# Autodesk Inventor assembly: 560H_plus_Blumotion NL=270 mm Chipboard screws 661.1450.HG 6,3x14,5 L Top row R Top row LD drillings both
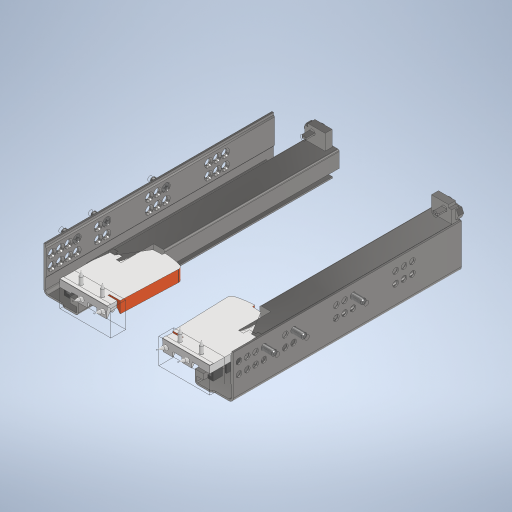
[picture p0: Inventor's stored thumbnail of the model, 512x512]
Saved by Autodesk Inventor 2024 (Build 280153000, 153)
## iProperties
Created: 2019-09-10
Part Number: 560H_plus_Blumotion NL=270 mm Chipboard screws 661.1450.HG 6,3x14,5 L Top row R Top row LD drillings both
Document SubType Name: Assembly
Designer: RokasM
Author: RokasM
## Documents named in this file (457)
- C:\W4INV 2024 Design\LIBRARY\Sliders\Blum TANDEM PLUS BLUMOTION 560 H\560H_iassembly_v2_LD.iam
- C:\W4INV 2024 Design\LIBRARY\Sliders\Blum TANDEM PLUS BLUMOTION 560 H\Blum_TANDEM_PLUS_BLUMOTION_560H.IPT
- C:\W4INV 2024 Design\LIBRARY\Sliders\Blum TANDEM PLUS BLUMOTION 560 H\Locking device.ipt
- C:\W4INV 2024 Design\LIBRARY\Sliders\Blum TANDEM PLUS BLUMOTION 560 H\Locking_device\Locking device L.ipt
- C:\W4INV 2024 Design\LIBRARY\Sliders\Blum TANDEM PLUS BLUMOTION 560 H\Locking_device\Locking device R.ipt
- C:\W4INV 2024 Design\LIBRARY\Sliders\Blum TANDEM PLUS BLUMOTION 560 H\560H\560H2700B Chipboard screws top_row L.ipt
- C:\W4INV 2024 Design\LIBRARY\Sliders\Blum TANDEM PLUS BLUMOTION 560 H\560H\560H2700B Chipboard screws top_row R.ipt
- C:\W4INV 2020 Design\LIBRARY\Rollers\Blum TANDEM PLUS BLUMOTION 560 H\Locking device.ipt
- 560H_plus_Blumotion NL=250 mm Chipboard screws 4x15 L Bottom row R Bottom row LD drillings B.iam
- 560H_plus_Blumotion NL=250 mm Chipboard screws 4x15 L Bottom row R Bottom row LD drillings both.iam
- 560H_plus_Blumotion NL=250 mm Chipboard screws 4x15 L Bottom row R Bottom row LD drillings F.iam
- 560H_plus_Blumotion NL=250 mm Chipboard screws 4x15 L Bottom row R Bottom row LD drillings none.iam
- 560H_plus_Blumotion NL=250 mm Chipboard screws 4x15 L Bottom row R Top row LD drillings B.iam
- 560H_plus_Blumotion NL=250 mm Chipboard screws 4x15 L Bottom row R Top row LD drillings both.iam
- 560H_plus_Blumotion NL=250 mm Chipboard screws 4x15 L Bottom row R Top row LD drillings F.iam
- 560H_plus_Blumotion NL=250 mm Chipboard screws 4x15 L Bottom row R Top row LD drillings none.iam
- 560H_plus_Blumotion NL=250 mm Chipboard screws 4x15 L Top row R Bottom row LD drillings B.iam
- 560H_plus_Blumotion NL=250 mm Chipboard screws 4x15 L Top row R Bottom row LD drillings both.iam
- 560H_plus_Blumotion NL=250 mm Chipboard screws 4x15 L Top row R Bottom row LD drillings F.iam
- 560H_plus_Blumotion NL=250 mm Chipboard screws 4x15 L Top row R Bottom row LD drillings none.iam
- 560H_plus_Blumotion NL=250 mm Chipboard screws 4x15 L Top row R Top row LD drillings B.iam
- 560H_plus_Blumotion NL=250 mm Chipboard screws 4x15 L Top row R Top row LD drillings both.iam
- 560H_plus_Blumotion NL=250 mm Chipboard screws 4x15 L Top row R Top row LD drillings F.iam
- 560H_plus_Blumotion NL=250 mm Chipboard screws 4x15 L Top row R Top row LD drillings none.iam
- 560H_plus_Blumotion NL=250 mm Chipboard screws 661.1450.HG 6,3x14,5 L Bottom row R Bottom row LD drillings B.iam
- 560H_plus_Blumotion NL=250 mm Chipboard screws 661.1450.HG 6,3x14,5 L Bottom row R Bottom row LD drillings both.iam
- 560H_plus_Blumotion NL=250 mm Chipboard screws 661.1450.HG 6,3x14,5 L Bottom row R Bottom row LD drillings F.iam
- 560H_plus_Blumotion NL=250 mm Chipboard screws 661.1450.HG 6,3x14,5 L Bottom row R Bottom row LD drillings none.iam
- 560H_plus_Blumotion NL=250 mm Chipboard screws 661.1450.HG 6,3x14,5 L Bottom row R Top row LD drillings B.iam
- 560H_plus_Blumotion NL=250 mm Chipboard screws 661.1450.HG 6,3x14,5 L Bottom row R Top row LD drillings both.iam
- 560H_plus_Blumotion NL=250 mm Chipboard screws 661.1450.HG 6,3x14,5 L Bottom row R Top row LD drillings F.iam
- 560H_plus_Blumotion NL=250 mm Chipboard screws 661.1450.HG 6,3x14,5 L Bottom row R Top row LD drillings none.iam
- 560H_plus_Blumotion NL=250 mm Chipboard screws 661.1450.HG 6,3x14,5 L Top row R Bottom row LD drillings B.iam
- 560H_plus_Blumotion NL=250 mm Chipboard screws 661.1450.HG 6,3x14,5 L Top row R Bottom row LD drillings both.iam
- 560H_plus_Blumotion NL=250 mm Chipboard screws 661.1450.HG 6,3x14,5 L Top row R Bottom row LD drillings F.iam
- 560H_plus_Blumotion NL=250 mm Chipboard screws 661.1450.HG 6,3x14,5 L Top row R Bottom row LD drillings none.iam
- 560H_plus_Blumotion NL=250 mm Chipboard screws 661.1450.HG 6,3x14,5 L Top row R Top row LD drillings B.iam
- 560H_plus_Blumotion NL=250 mm Chipboard screws 661.1450.HG 6,3x14,5 L Top row R Top row LD drillings both.iam
- 560H_plus_Blumotion NL=250 mm Chipboard screws 661.1450.HG 6,3x14,5 L Top row R Top row LD drillings F.iam
- 560H_plus_Blumotion NL=250 mm Chipboard screws 661.1450.HG 6,3x14,5 L Top row R Top row LD drillings none.iam
- 560H_plus_Blumotion NL=270 mm Chipboard screws 4x15 L Bottom row R Bottom row LD drillings B.iam
- 560H_plus_Blumotion NL=270 mm Chipboard screws 4x15 L Bottom row R Bottom row LD drillings both.iam
- 560H_plus_Blumotion NL=270 mm Chipboard screws 4x15 L Bottom row R Bottom row LD drillings F.iam
- 560H_plus_Blumotion NL=270 mm Chipboard screws 4x15 L Bottom row R Bottom row LD drillings none.iam
- 560H_plus_Blumotion NL=270 mm Chipboard screws 4x15 L Bottom row R Top row LD drillings B.iam
- 560H_plus_Blumotion NL=270 mm Chipboard screws 4x15 L Bottom row R Top row LD drillings both.iam
- 560H_plus_Blumotion NL=270 mm Chipboard screws 4x15 L Bottom row R Top row LD drillings F.iam
- 560H_plus_Blumotion NL=270 mm Chipboard screws 4x15 L Bottom row R Top row LD drillings none.iam
- 560H_plus_Blumotion NL=270 mm Chipboard screws 4x15 L Top row R Bottom row LD drillings B.iam
- 560H_plus_Blumotion NL=270 mm Chipboard screws 4x15 L Top row R Bottom row LD drillings both.iam
- 560H_plus_Blumotion NL=270 mm Chipboard screws 4x15 L Top row R Bottom row LD drillings F.iam
- 560H_plus_Blumotion NL=270 mm Chipboard screws 4x15 L Top row R Bottom row LD drillings none.iam
- 560H_plus_Blumotion NL=270 mm Chipboard screws 4x15 L Top row R Top row LD drillings B.iam
- 560H_plus_Blumotion NL=270 mm Chipboard screws 4x15 L Top row R Top row LD drillings both.iam
- 560H_plus_Blumotion NL=270 mm Chipboard screws 4x15 L Top row R Top row LD drillings F.iam
- 560H_plus_Blumotion NL=270 mm Chipboard screws 4x15 L Top row R Top row LD drillings none.iam
- 560H_plus_Blumotion NL=270 mm Chipboard screws 661.1450.HG 6,3x14,5 L Bottom row R Bottom row LD drillings B.iam
- 560H_plus_Blumotion NL=270 mm Chipboard screws 661.1450.HG 6,3x14,5 L Bottom row R Bottom row LD drillings both.iam
- 560H_plus_Blumotion NL=270 mm Chipboard screws 661.1450.HG 6,3x14,5 L Bottom row R Bottom row LD drillings F.iam
- 560H_plus_Blumotion NL=270 mm Chipboard screws 661.1450.HG 6,3x14,5 L Bottom row R Bottom row LD drillings none.iam
- 560H_plus_Blumotion NL=270 mm Chipboard screws 661.1450.HG 6,3x14,5 L Bottom row R Top row LD drillings B.iam
- 560H_plus_Blumotion NL=270 mm Chipboard screws 661.1450.HG 6,3x14,5 L Bottom row R Top row LD drillings both.iam
- 560H_plus_Blumotion NL=270 mm Chipboard screws 661.1450.HG 6,3x14,5 L Bottom row R Top row LD drillings F.iam
- 560H_plus_Blumotion NL=270 mm Chipboard screws 661.1450.HG 6,3x14,5 L Bottom row R Top row LD drillings none.iam
- 560H_plus_Blumotion NL=270 mm Chipboard screws 661.1450.HG 6,3x14,5 L Top row R Bottom row LD drillings B.iam
- 560H_plus_Blumotion NL=270 mm Chipboard screws 661.1450.HG 6,3x14,5 L Top row R Bottom row LD drillings both.iam
- 560H_plus_Blumotion NL=270 mm Chipboard screws 661.1450.HG 6,3x14,5 L Top row R Bottom row LD drillings F.iam
- 560H_plus_Blumotion NL=270 mm Chipboard screws 661.1450.HG 6,3x14,5 L Top row R Bottom row LD drillings none.iam
- 560H_plus_Blumotion NL=270 mm Chipboard screws 661.1450.HG 6,3x14,5 L Top row R Top row LD drillings B.iam
- 560H_plus_Blumotion NL=270 mm Chipboard screws 661.1450.HG 6,3x14,5 L Top row R Top row LD drillings both.iam
- 560H_plus_Blumotion NL=270 mm Chipboard screws 661.1450.HG 6,3x14,5 L Top row R Top row LD drillings F.iam
- 560H_plus_Blumotion NL=270 mm Chipboard screws 661.1450.HG 6,3x14,5 L Top row R Top row LD drillings none.iam
- 560H_plus_Blumotion NL=300 mm Chipboard screws 4x15 L Bottom row R Bottom row LD drillings B.iam
- 560H_plus_Blumotion NL=300 mm Chipboard screws 4x15 L Bottom row R Bottom row LD drillings both.iam
- 560H_plus_Blumotion NL=300 mm Chipboard screws 4x15 L Bottom row R Bottom row LD drillings F.iam
- 560H_plus_Blumotion NL=300 mm Chipboard screws 4x15 L Bottom row R Bottom row LD drillings none.iam
- 560H_plus_Blumotion NL=300 mm Chipboard screws 4x15 L Bottom row R Top row LD drillings B.iam
- 560H_plus_Blumotion NL=300 mm Chipboard screws 4x15 L Bottom row R Top row LD drillings both.iam
- 560H_plus_Blumotion NL=300 mm Chipboard screws 4x15 L Bottom row R Top row LD drillings F.iam
- 560H_plus_Blumotion NL=300 mm Chipboard screws 4x15 L Bottom row R Top row LD drillings none.iam
- 560H_plus_Blumotion NL=300 mm Chipboard screws 4x15 L Top row R Bottom row LD drillings B.iam
- 560H_plus_Blumotion NL=300 mm Chipboard screws 4x15 L Top row R Bottom row LD drillings both.iam
- 560H_plus_Blumotion NL=300 mm Chipboard screws 4x15 L Top row R Bottom row LD drillings F.iam
- 560H_plus_Blumotion NL=300 mm Chipboard screws 4x15 L Top row R Bottom row LD drillings none.iam
- 560H_plus_Blumotion NL=300 mm Chipboard screws 4x15 L Top row R Top row LD drillings B.iam
- 560H_plus_Blumotion NL=300 mm Chipboard screws 4x15 L Top row R Top row LD drillings both.iam
- 560H_plus_Blumotion NL=300 mm Chipboard screws 4x15 L Top row R Top row LD drillings F.iam
- 560H_plus_Blumotion NL=300 mm Chipboard screws 4x15 L Top row R Top row LD drillings none.iam
- 560H_plus_Blumotion NL=300 mm Chipboard screws 661.1450.HG 6,3x14,5 L Bottom row R Bottom row LD drillings B.iam
- 560H_plus_Blumotion NL=300 mm Chipboard screws 661.1450.HG 6,3x14,5 L Bottom row R Bottom row LD drillings both.iam
- 560H_plus_Blumotion NL=300 mm Chipboard screws 661.1450.HG 6,3x14,5 L Bottom row R Bottom row LD drillings F.iam
- 560H_plus_Blumotion NL=300 mm Chipboard screws 661.1450.HG 6,3x14,5 L Bottom row R Bottom row LD drillings none.iam
- 560H_plus_Blumotion NL=300 mm Chipboard screws 661.1450.HG 6,3x14,5 L Bottom row R Top row LD drillings B.iam
- 560H_plus_Blumotion NL=300 mm Chipboard screws 661.1450.HG 6,3x14,5 L Bottom row R Top row LD drillings both.iam
- 560H_plus_Blumotion NL=300 mm Chipboard screws 661.1450.HG 6,3x14,5 L Bottom row R Top row LD drillings F.iam
- 560H_plus_Blumotion NL=300 mm Chipboard screws 661.1450.HG 6,3x14,5 L Bottom row R Top row LD drillings none.iam
- 560H_plus_Blumotion NL=300 mm Chipboard screws 661.1450.HG 6,3x14,5 L Top row R Bottom row LD drillings B.iam
- 560H_plus_Blumotion NL=300 mm Chipboard screws 661.1450.HG 6,3x14,5 L Top row R Bottom row LD drillings both.iam
- 560H_plus_Blumotion NL=300 mm Chipboard screws 661.1450.HG 6,3x14,5 L Top row R Bottom row LD drillings F.iam
- 560H_plus_Blumotion NL=300 mm Chipboard screws 661.1450.HG 6,3x14,5 L Top row R Bottom row LD drillings none.iam
- 560H_plus_Blumotion NL=300 mm Chipboard screws 661.1450.HG 6,3x14,5 L Top row R Top row LD drillings B.iam
- 560H_plus_Blumotion NL=300 mm Chipboard screws 661.1450.HG 6,3x14,5 L Top row R Top row LD drillings both.iam
- 560H_plus_Blumotion NL=300 mm Chipboard screws 661.1450.HG 6,3x14,5 L Top row R Top row LD drillings F.iam
- 560H_plus_Blumotion NL=300 mm Chipboard screws 661.1450.HG 6,3x14,5 L Top row R Top row LD drillings none.iam
- 560H_plus_Blumotion NL=320 mm Chipboard screws 4x15 L Bottom row R Bottom row LD drillings B.iam
- 560H_plus_Blumotion NL=320 mm Chipboard screws 4x15 L Bottom row R Bottom row LD drillings both.iam
- 560H_plus_Blumotion NL=320 mm Chipboard screws 4x15 L Bottom row R Bottom row LD drillings F.iam
- 560H_plus_Blumotion NL=320 mm Chipboard screws 4x15 L Bottom row R Bottom row LD drillings none.iam
- 560H_plus_Blumotion NL=320 mm Chipboard screws 4x15 L Bottom row R Top row LD drillings B.iam
- 560H_plus_Blumotion NL=320 mm Chipboard screws 4x15 L Bottom row R Top row LD drillings both.iam
- 560H_plus_Blumotion NL=320 mm Chipboard screws 4x15 L Bottom row R Top row LD drillings F.iam
- 560H_plus_Blumotion NL=320 mm Chipboard screws 4x15 L Bottom row R Top row LD drillings none.iam
- 560H_plus_Blumotion NL=320 mm Chipboard screws 4x15 L Top row R Bottom row LD drillings B.iam
- 560H_plus_Blumotion NL=320 mm Chipboard screws 4x15 L Top row R Bottom row LD drillings both.iam
- 560H_plus_Blumotion NL=320 mm Chipboard screws 4x15 L Top row R Bottom row LD drillings F.iam
- 560H_plus_Blumotion NL=320 mm Chipboard screws 4x15 L Top row R Bottom row LD drillings none.iam
- 560H_plus_Blumotion NL=320 mm Chipboard screws 4x15 L Top row R Top row LD drillings B.iam
- 560H_plus_Blumotion NL=320 mm Chipboard screws 4x15 L Top row R Top row LD drillings both.iam
- 560H_plus_Blumotion NL=320 mm Chipboard screws 4x15 L Top row R Top row LD drillings F.iam
- 560H_plus_Blumotion NL=320 mm Chipboard screws 4x15 L Top row R Top row LD drillings none.iam
- 560H_plus_Blumotion NL=320 mm Chipboard screws 661.1450.HG 6,3x14,5 L Bottom row R Bottom row LD drillings B.iam
- 560H_plus_Blumotion NL=320 mm Chipboard screws 661.1450.HG 6,3x14,5 L Bottom row R Bottom row LD drillings both.iam
- 560H_plus_Blumotion NL=320 mm Chipboard screws 661.1450.HG 6,3x14,5 L Bottom row R Bottom row LD drillings F.iam
- 560H_plus_Blumotion NL=320 mm Chipboard screws 661.1450.HG 6,3x14,5 L Bottom row R Bottom row LD drillings none.iam
- 560H_plus_Blumotion NL=320 mm Chipboard screws 661.1450.HG 6,3x14,5 L Bottom row R Top row LD drillings B.iam
- 560H_plus_Blumotion NL=320 mm Chipboard screws 661.1450.HG 6,3x14,5 L Bottom row R Top row LD drillings both.iam
- 560H_plus_Blumotion NL=320 mm Chipboard screws 661.1450.HG 6,3x14,5 L Bottom row R Top row LD drillings F.iam
- 560H_plus_Blumotion NL=320 mm Chipboard screws 661.1450.HG 6,3x14,5 L Bottom row R Top row LD drillings none.iam
- 560H_plus_Blumotion NL=320 mm Chipboard screws 661.1450.HG 6,3x14,5 L Top row R Bottom row LD drillings B.iam
- 560H_plus_Blumotion NL=320 mm Chipboard screws 661.1450.HG 6,3x14,5 L Top row R Bottom row LD drillings both.iam
- 560H_plus_Blumotion NL=320 mm Chipboard screws 661.1450.HG 6,3x14,5 L Top row R Bottom row LD drillings F.iam
- 560H_plus_Blumotion NL=320 mm Chipboard screws 661.1450.HG 6,3x14,5 L Top row R Bottom row LD drillings none.iam
- 560H_plus_Blumotion NL=320 mm Chipboard screws 661.1450.HG 6,3x14,5 L Top row R Top row LD drillings B.iam
- 560H_plus_Blumotion NL=320 mm Chipboard screws 661.1450.HG 6,3x14,5 L Top row R Top row LD drillings both.iam
- 560H_plus_Blumotion NL=320 mm Chipboard screws 661.1450.HG 6,3x14,5 L Top row R Top row LD drillings F.iam
- 560H_plus_Blumotion NL=320 mm Chipboard screws 661.1450.HG 6,3x14,5 L Top row R Top row LD drillings none.iam
- 560H_plus_Blumotion NL=350 mm Chipboard screws 4x15 L Bottom row R Bottom row LD drillings B.iam
- 560H_plus_Blumotion NL=350 mm Chipboard screws 4x15 L Bottom row R Bottom row LD drillings both.iam
- 560H_plus_Blumotion NL=350 mm Chipboard screws 4x15 L Bottom row R Bottom row LD drillings F.iam
- 560H_plus_Blumotion NL=350 mm Chipboard screws 4x15 L Bottom row R Bottom row LD drillings none.iam
- 560H_plus_Blumotion NL=350 mm Chipboard screws 4x15 L Bottom row R Top row LD drillings B.iam
- 560H_plus_Blumotion NL=350 mm Chipboard screws 4x15 L Bottom row R Top row LD drillings both.iam
- 560H_plus_Blumotion NL=350 mm Chipboard screws 4x15 L Bottom row R Top row LD drillings F.iam
- 560H_plus_Blumotion NL=350 mm Chipboard screws 4x15 L Bottom row R Top row LD drillings none.iam
- 560H_plus_Blumotion NL=350 mm Chipboard screws 4x15 L Top row R Bottom row LD drillings B.iam
- 560H_plus_Blumotion NL=350 mm Chipboard screws 4x15 L Top row R Bottom row LD drillings both.iam
- 560H_plus_Blumotion NL=350 mm Chipboard screws 4x15 L Top row R Bottom row LD drillings F.iam
- 560H_plus_Blumotion NL=350 mm Chipboard screws 4x15 L Top row R Bottom row LD drillings none.iam
- 560H_plus_Blumotion NL=350 mm Chipboard screws 4x15 L Top row R Top row LD drillings B.iam
- 560H_plus_Blumotion NL=350 mm Chipboard screws 4x15 L Top row R Top row LD drillings both.iam
- 560H_plus_Blumotion NL=350 mm Chipboard screws 4x15 L Top row R Top row LD drillings F.iam
- 560H_plus_Blumotion NL=350 mm Chipboard screws 4x15 L Top row R Top row LD drillings none.iam
- 560H_plus_Blumotion NL=350 mm Chipboard screws 661.1450.HG 6,3x14,5 L Bottom row R Bottom row LD drillings B.iam
- 560H_plus_Blumotion NL=350 mm Chipboard screws 661.1450.HG 6,3x14,5 L Bottom row R Bottom row LD drillings both.iam
- 560H_plus_Blumotion NL=350 mm Chipboard screws 661.1450.HG 6,3x14,5 L Bottom row R Bottom row LD drillings F.iam
- 560H_plus_Blumotion NL=350 mm Chipboard screws 661.1450.HG 6,3x14,5 L Bottom row R Bottom row LD drillings none.iam
- 560H_plus_Blumotion NL=350 mm Chipboard screws 661.1450.HG 6,3x14,5 L Bottom row R Top row LD drillings B.iam
- 560H_plus_Blumotion NL=350 mm Chipboard screws 661.1450.HG 6,3x14,5 L Bottom row R Top row LD drillings both.iam
- 560H_plus_Blumotion NL=350 mm Chipboard screws 661.1450.HG 6,3x14,5 L Bottom row R Top row LD drillings F.iam
- 560H_plus_Blumotion NL=350 mm Chipboard screws 661.1450.HG 6,3x14,5 L Bottom row R Top row LD drillings none.iam
- 560H_plus_Blumotion NL=350 mm Chipboard screws 661.1450.HG 6,3x14,5 L Top row R Bottom row LD drillings B.iam
- 560H_plus_Blumotion NL=350 mm Chipboard screws 661.1450.HG 6,3x14,5 L Top row R Bottom row LD drillings both.iam
- 560H_plus_Blumotion NL=350 mm Chipboard screws 661.1450.HG 6,3x14,5 L Top row R Bottom row LD drillings F.iam
- 560H_plus_Blumotion NL=350 mm Chipboard screws 661.1450.HG 6,3x14,5 L Top row R Bottom row LD drillings none.iam
- 560H_plus_Blumotion NL=350 mm Chipboard screws 661.1450.HG 6,3x14,5 L Top row R Top row LD drillings B.iam
- 560H_plus_Blumotion NL=350 mm Chipboard screws 661.1450.HG 6,3x14,5 L Top row R Top row LD drillings both.iam
- 560H_plus_Blumotion NL=350 mm Chipboard screws 661.1450.HG 6,3x14,5 L Top row R Top row LD drillings F.iam
- 560H_plus_Blumotion NL=350 mm Chipboard screws 661.1450.HG 6,3x14,5 L Top row R Top row LD drillings none.iam
- 560H_plus_Blumotion NL=380 mm Chipboard screws 4x15 L Bottom row R Bottom row LD drillings B.iam
- 560H_plus_Blumotion NL=380 mm Chipboard screws 4x15 L Bottom row R Bottom row LD drillings both.iam
- 560H_plus_Blumotion NL=380 mm Chipboard screws 4x15 L Bottom row R Bottom row LD drillings F.iam
- 560H_plus_Blumotion NL=380 mm Chipboard screws 4x15 L Bottom row R Bottom row LD drillings none.iam
- 560H_plus_Blumotion NL=380 mm Chipboard screws 4x15 L Bottom row R Top row LD drillings B.iam
- 560H_plus_Blumotion NL=380 mm Chipboard screws 4x15 L Bottom row R Top row LD drillings both.iam
- 560H_plus_Blumotion NL=380 mm Chipboard screws 4x15 L Bottom row R Top row LD drillings F.iam
- 560H_plus_Blumotion NL=380 mm Chipboard screws 4x15 L Bottom row R Top row LD drillings none.iam
- 560H_plus_Blumotion NL=380 mm Chipboard screws 4x15 L Top row R Bottom row LD drillings B.iam
- 560H_plus_Blumotion NL=380 mm Chipboard screws 4x15 L Top row R Bottom row LD drillings both.iam
- 560H_plus_Blumotion NL=380 mm Chipboard screws 4x15 L Top row R Bottom row LD drillings F.iam
- 560H_plus_Blumotion NL=380 mm Chipboard screws 4x15 L Top row R Bottom row LD drillings none.iam
- 560H_plus_Blumotion NL=380 mm Chipboard screws 4x15 L Top row R Top row LD drillings B.iam
- 560H_plus_Blumotion NL=380 mm Chipboard screws 4x15 L Top row R Top row LD drillings both.iam
- 560H_plus_Blumotion NL=380 mm Chipboard screws 4x15 L Top row R Top row LD drillings F.iam
- 560H_plus_Blumotion NL=380 mm Chipboard screws 4x15 L Top row R Top row LD drillings none.iam
- 560H_plus_Blumotion NL=380 mm Chipboard screws 661.1450.HG 6,3x14,5 L Bottom row R Bottom row LD drillings B.iam
- 560H_plus_Blumotion NL=380 mm Chipboard screws 661.1450.HG 6,3x14,5 L Bottom row R Bottom row LD drillings both.iam
- 560H_plus_Blumotion NL=380 mm Chipboard screws 661.1450.HG 6,3x14,5 L Bottom row R Bottom row LD drillings F.iam
- 560H_plus_Blumotion NL=380 mm Chipboard screws 661.1450.HG 6,3x14,5 L Bottom row R Bottom row LD drillings none.iam
- 560H_plus_Blumotion NL=380 mm Chipboard screws 661.1450.HG 6,3x14,5 L Bottom row R Top row LD drillings B.iam
- 560H_plus_Blumotion NL=380 mm Chipboard screws 661.1450.HG 6,3x14,5 L Bottom row R Top row LD drillings both.iam
- 560H_plus_Blumotion NL=380 mm Chipboard screws 661.1450.HG 6,3x14,5 L Bottom row R Top row LD drillings F.iam
- 560H_plus_Blumotion NL=380 mm Chipboard screws 661.1450.HG 6,3x14,5 L Bottom row R Top row LD drillings none.iam
- 560H_plus_Blumotion NL=380 mm Chipboard screws 661.1450.HG 6,3x14,5 L Top row R Bottom row LD drillings B.iam
- 560H_plus_Blumotion NL=380 mm Chipboard screws 661.1450.HG 6,3x14,5 L Top row R Bottom row LD drillings both.iam
- 560H_plus_Blumotion NL=380 mm Chipboard screws 661.1450.HG 6,3x14,5 L Top row R Bottom row LD drillings F.iam
- 560H_plus_Blumotion NL=380 mm Chipboard screws 661.1450.HG 6,3x14,5 L Top row R Bottom row LD drillings none.iam
- 560H_plus_Blumotion NL=380 mm Chipboard screws 661.1450.HG 6,3x14,5 L Top row R Top row LD drillings B.iam
- 560H_plus_Blumotion NL=380 mm Chipboard screws 661.1450.HG 6,3x14,5 L Top row R Top row LD drillings both.iam
- 560H_plus_Blumotion NL=380 mm Chipboard screws 661.1450.HG 6,3x14,5 L Top row R Top row LD drillings F.iam
- 560H_plus_Blumotion NL=380 mm Chipboard screws 661.1450.HG 6,3x14,5 L Top row R Top row LD drillings none.iam
- 560H_plus_Blumotion NL=400 mm Chipboard screws 4x15 L Bottom row R Bottom row LD drillings B.iam
- 560H_plus_Blumotion NL=400 mm Chipboard screws 4x15 L Bottom row R Bottom row LD drillings both.iam
- 560H_plus_Blumotion NL=400 mm Chipboard screws 4x15 L Bottom row R Bottom row LD drillings F.iam
- 560H_plus_Blumotion NL=400 mm Chipboard screws 4x15 L Bottom row R Bottom row LD drillings none.iam
- 560H_plus_Blumotion NL=400 mm Chipboard screws 4x15 L Bottom row R Top row LD drillings B.iam
- 560H_plus_Blumotion NL=400 mm Chipboard screws 4x15 L Bottom row R Top row LD drillings both.iam
- 560H_plus_Blumotion NL=400 mm Chipboard screws 4x15 L Bottom row R Top row LD drillings F.iam
- 560H_plus_Blumotion NL=400 mm Chipboard screws 4x15 L Bottom row R Top row LD drillings none.iam
- 560H_plus_Blumotion NL=400 mm Chipboard screws 4x15 L Top row R Bottom row LD drillings B.iam
- 560H_plus_Blumotion NL=400 mm Chipboard screws 4x15 L Top row R Bottom row LD drillings both.iam
- 560H_plus_Blumotion NL=400 mm Chipboard screws 4x15 L Top row R Bottom row LD drillings F.iam
- 560H_plus_Blumotion NL=400 mm Chipboard screws 4x15 L Top row R Bottom row LD drillings none.iam
- 560H_plus_Blumotion NL=400 mm Chipboard screws 4x15 L Top row R Top row LD drillings B.iam
- 560H_plus_Blumotion NL=400 mm Chipboard screws 4x15 L Top row R Top row LD drillings both.iam
- 560H_plus_Blumotion NL=400 mm Chipboard screws 4x15 L Top row R Top row LD drillings F.iam
- 560H_plus_Blumotion NL=400 mm Chipboard screws 4x15 L Top row R Top row LD drillings none.iam
- 560H_plus_Blumotion NL=400 mm Chipboard screws 661.1450.HG 6,3x14,5 L Bottom row R Bottom row LD drillings B.iam
- 560H_plus_Blumotion NL=400 mm Chipboard screws 661.1450.HG 6,3x14,5 L Bottom row R Bottom row LD drillings both.iam
- 560H_plus_Blumotion NL=400 mm Chipboard screws 661.1450.HG 6,3x14,5 L Bottom row R Bottom row LD drillings F.iam
- 560H_plus_Blumotion NL=400 mm Chipboard screws 661.1450.HG 6,3x14,5 L Bottom row R Bottom row LD drillings none.iam
- 560H_plus_Blumotion NL=400 mm Chipboard screws 661.1450.HG 6,3x14,5 L Bottom row R Top row LD drillings B.iam
- 560H_plus_Blumotion NL=400 mm Chipboard screws 661.1450.HG 6,3x14,5 L Bottom row R Top row LD drillings both.iam
- 560H_plus_Blumotion NL=400 mm Chipboard screws 661.1450.HG 6,3x14,5 L Bottom row R Top row LD drillings F.iam
- 560H_plus_Blumotion NL=400 mm Chipboard screws 661.1450.HG 6,3x14,5 L Bottom row R Top row LD drillings none.iam
- 560H_plus_Blumotion NL=400 mm Chipboard screws 661.1450.HG 6,3x14,5 L Top row R Bottom row LD drillings B.iam
- 560H_plus_Blumotion NL=400 mm Chipboard screws 661.1450.HG 6,3x14,5 L Top row R Bottom row LD drillings both.iam
- 560H_plus_Blumotion NL=400 mm Chipboard screws 661.1450.HG 6,3x14,5 L Top row R Bottom row LD drillings F.iam
- 560H_plus_Blumotion NL=400 mm Chipboard screws 661.1450.HG 6,3x14,5 L Top row R Bottom row LD drillings none.iam
- 560H_plus_Blumotion NL=400 mm Chipboard screws 661.1450.HG 6,3x14,5 L Top row R Top row LD drillings B.iam
- 560H_plus_Blumotion NL=400 mm Chipboard screws 661.1450.HG 6,3x14,5 L Top row R Top row LD drillings both.iam
- 560H_plus_Blumotion NL=400 mm Chipboard screws 661.1450.HG 6,3x14,5 L Top row R Top row LD drillings F.iam
- 560H_plus_Blumotion NL=400 mm Chipboard screws 661.1450.HG 6,3x14,5 L Top row R Top row LD drillings none.iam
- 560H_plus_Blumotion NL=420 mm Chipboard screws 4x15 L Bottom row R Bottom row LD drillings B.iam
- 560H_plus_Blumotion NL=420 mm Chipboard screws 4x15 L Bottom row R Bottom row LD drillings both.iam
- 560H_plus_Blumotion NL=420 mm Chipboard screws 4x15 L Bottom row R Bottom row LD drillings F.iam
- 560H_plus_Blumotion NL=420 mm Chipboard screws 4x15 L Bottom row R Bottom row LD drillings none.iam
- 560H_plus_Blumotion NL=420 mm Chipboard screws 4x15 L Bottom row R Top row LD drillings B.iam
- 560H_plus_Blumotion NL=420 mm Chipboard screws 4x15 L Bottom row R Top row LD drillings both.iam
- 560H_plus_Blumotion NL=420 mm Chipboard screws 4x15 L Bottom row R Top row LD drillings F.iam
- 560H_plus_Blumotion NL=420 mm Chipboard screws 4x15 L Bottom row R Top row LD drillings none.iam
- 560H_plus_Blumotion NL=420 mm Chipboard screws 4x15 L Top row R Bottom row LD drillings B.iam
- 560H_plus_Blumotion NL=420 mm Chipboard screws 4x15 L Top row R Bottom row LD drillings both.iam
- 560H_plus_Blumotion NL=420 mm Chipboard screws 4x15 L Top row R Bottom row LD drillings F.iam
- 560H_plus_Blumotion NL=420 mm Chipboard screws 4x15 L Top row R Bottom row LD drillings none.iam
- 560H_plus_Blumotion NL=420 mm Chipboard screws 4x15 L Top row R Top row LD drillings B.iam
- 560H_plus_Blumotion NL=420 mm Chipboard screws 4x15 L Top row R Top row LD drillings both.iam
- 560H_plus_Blumotion NL=420 mm Chipboard screws 4x15 L Top row R Top row LD drillings F.iam
- 560H_plus_Blumotion NL=420 mm Chipboard screws 4x15 L Top row R Top row LD drillings none.iam
- 560H_plus_Blumotion NL=420 mm Chipboard screws 661.1450.HG 6,3x14,5 L Bottom row R Bottom row LD drillings B.iam
- 560H_plus_Blumotion NL=420 mm Chipboard screws 661.1450.HG 6,3x14,5 L Bottom row R Bottom row LD drillings both.iam
- 560H_plus_Blumotion NL=420 mm Chipboard screws 661.1450.HG 6,3x14,5 L Bottom row R Bottom row LD drillings F.iam
- 560H_plus_Blumotion NL=420 mm Chipboard screws 661.1450.HG 6,3x14,5 L Bottom row R Bottom row LD drillings none.iam
- 560H_plus_Blumotion NL=420 mm Chipboard screws 661.1450.HG 6,3x14,5 L Bottom row R Top row LD drillings B.iam
- 560H_plus_Blumotion NL=420 mm Chipboard screws 661.1450.HG 6,3x14,5 L Bottom row R Top row LD drillings both.iam
- 560H_plus_Blumotion NL=420 mm Chipboard screws 661.1450.HG 6,3x14,5 L Bottom row R Top row LD drillings F.iam
- 560H_plus_Blumotion NL=420 mm Chipboard screws 661.1450.HG 6,3x14,5 L Bottom row R Top row LD drillings none.iam
- 560H_plus_Blumotion NL=420 mm Chipboard screws 661.1450.HG 6,3x14,5 L Top row R Bottom row LD drillings B.iam
- 560H_plus_Blumotion NL=420 mm Chipboard screws 661.1450.HG 6,3x14,5 L Top row R Bottom row LD drillings both.iam
- 560H_plus_Blumotion NL=420 mm Chipboard screws 661.1450.HG 6,3x14,5 L Top row R Bottom row LD drillings F.iam
- 560H_plus_Blumotion NL=420 mm Chipboard screws 661.1450.HG 6,3x14,5 L Top row R Bottom row LD drillings none.iam
- 560H_plus_Blumotion NL=420 mm Chipboard screws 661.1450.HG 6,3x14,5 L Top row R Top row LD drillings B.iam
- 560H_plus_Blumotion NL=420 mm Chipboard screws 661.1450.HG 6,3x14,5 L Top row R Top row LD drillings both.iam
- 560H_plus_Blumotion NL=420 mm Chipboard screws 661.1450.HG 6,3x14,5 L Top row R Top row LD drillings F.iam
- 560H_plus_Blumotion NL=420 mm Chipboard screws 661.1450.HG 6,3x14,5 L Top row R Top row LD drillings none.iam
- 560H_plus_Blumotion NL=450 mm Chipboard screws 4x15 L Bottom row R Bottom row LD drillings B.iam
- 560H_plus_Blumotion NL=450 mm Chipboard screws 4x15 L Bottom row R Bottom row LD drillings both.iam
- 560H_plus_Blumotion NL=450 mm Chipboard screws 4x15 L Bottom row R Bottom row LD drillings F.iam
- 560H_plus_Blumotion NL=450 mm Chipboard screws 4x15 L Bottom row R Bottom row LD drillings none.iam
- 560H_plus_Blumotion NL=450 mm Chipboard screws 4x15 L Bottom row R Top row LD drillings B.iam
- 560H_plus_Blumotion NL=450 mm Chipboard screws 4x15 L Bottom row R Top row LD drillings both.iam
- 560H_plus_Blumotion NL=450 mm Chipboard screws 4x15 L Bottom row R Top row LD drillings F.iam
- 560H_plus_Blumotion NL=450 mm Chipboard screws 4x15 L Bottom row R Top row LD drillings none.iam
- 560H_plus_Blumotion NL=450 mm Chipboard screws 4x15 L Top row R Bottom row LD drillings B.iam
- 560H_plus_Blumotion NL=450 mm Chipboard screws 4x15 L Top row R Bottom row LD drillings both.iam
- 560H_plus_Blumotion NL=450 mm Chipboard screws 4x15 L Top row R Bottom row LD drillings F.iam
- 560H_plus_Blumotion NL=450 mm Chipboard screws 4x15 L Top row R Bottom row LD drillings none.iam
- 560H_plus_Blumotion NL=450 mm Chipboard screws 4x15 L Top row R Top row LD drillings B.iam
- 560H_plus_Blumotion NL=450 mm Chipboard screws 4x15 L Top row R Top row LD drillings both.iam
- 560H_plus_Blumotion NL=450 mm Chipboard screws 4x15 L Top row R Top row LD drillings F.iam
- 560H_plus_Blumotion NL=450 mm Chipboard screws 4x15 L Top row R Top row LD drillings none.iam
- 560H_plus_Blumotion NL=450 mm Chipboard screws 661.1450.HG 6,3x14,5 L Bottom row R Bottom row LD drillings B.iam
- 560H_plus_Blumotion NL=450 mm Chipboard screws 661.1450.HG 6,3x14,5 L Bottom row R Bottom row LD drillings both.iam
- 560H_plus_Blumotion NL=450 mm Chipboard screws 661.1450.HG 6,3x14,5 L Bottom row R Bottom row LD drillings F.iam
- 560H_plus_Blumotion NL=450 mm Chipboard screws 661.1450.HG 6,3x14,5 L Bottom row R Bottom row LD drillings none.iam
- 560H_plus_Blumotion NL=450 mm Chipboard screws 661.1450.HG 6,3x14,5 L Bottom row R Top row LD drillings B.iam
- 560H_plus_Blumotion NL=450 mm Chipboard screws 661.1450.HG 6,3x14,5 L Bottom row R Top row LD drillings both.iam
- 560H_plus_Blumotion NL=450 mm Chipboard screws 661.1450.HG 6,3x14,5 L Bottom row R Top row LD drillings F.iam
- 560H_plus_Blumotion NL=450 mm Chipboard screws 661.1450.HG 6,3x14,5 L Bottom row R Top row LD drillings none.iam
- 560H_plus_Blumotion NL=450 mm Chipboard screws 661.1450.HG 6,3x14,5 L Top row R Bottom row LD drillings B.iam
- 560H_plus_Blumotion NL=450 mm Chipboard screws 661.1450.HG 6,3x14,5 L Top row R Bottom row LD drillings both.iam
- 560H_plus_Blumotion NL=450 mm Chipboard screws 661.1450.HG 6,3x14,5 L Top row R Bottom row LD drillings F.iam
- 560H_plus_Blumotion NL=450 mm Chipboard screws 661.1450.HG 6,3x14,5 L Top row R Bottom row LD drillings none.iam
- 560H_plus_Blumotion NL=450 mm Chipboard screws 661.1450.HG 6,3x14,5 L Top row R Top row LD drillings B.iam
- 560H_plus_Blumotion NL=450 mm Chipboard screws 661.1450.HG 6,3x14,5 L Top row R Top row LD drillings both.iam
- 560H_plus_Blumotion NL=450 mm Chipboard screws 661.1450.HG 6,3x14,5 L Top row R Top row LD drillings F.iam
- 560H_plus_Blumotion NL=450 mm Chipboard screws 661.1450.HG 6,3x14,5 L Top row R Top row LD drillings none.iam
- 560H_plus_Blumotion NL=480 mm Chipboard screws 4x15 L Bottom row R Bottom row LD drillings B.iam
- 560H_plus_Blumotion NL=480 mm Chipboard screws 4x15 L Bottom row R Bottom row LD drillings both.iam
- 560H_plus_Blumotion NL=480 mm Chipboard screws 4x15 L Bottom row R Bottom row LD drillings F.iam
- 560H_plus_Blumotion NL=480 mm Chipboard screws 4x15 L Bottom row R Bottom row LD drillings none.iam
- 560H_plus_Blumotion NL=480 mm Chipboard screws 4x15 L Bottom row R Top row LD drillings B.iam
- 560H_plus_Blumotion NL=480 mm Chipboard screws 4x15 L Bottom row R Top row LD drillings both.iam
- 560H_plus_Blumotion NL=480 mm Chipboard screws 4x15 L Bottom row R Top row LD drillings F.iam
- 560H_plus_Blumotion NL=480 mm Chipboard screws 4x15 L Bottom row R Top row LD drillings none.iam
- 560H_plus_Blumotion NL=480 mm Chipboard screws 4x15 L Top row R Bottom row LD drillings B.iam
- 560H_plus_Blumotion NL=480 mm Chipboard screws 4x15 L Top row R Bottom row LD drillings both.iam
- 560H_plus_Blumotion NL=480 mm Chipboard screws 4x15 L Top row R Bottom row LD drillings F.iam
- 560H_plus_Blumotion NL=480 mm Chipboard screws 4x15 L Top row R Bottom row LD drillings none.iam
- 560H_plus_Blumotion NL=480 mm Chipboard screws 4x15 L Top row R Top row LD drillings B.iam
- 560H_plus_Blumotion NL=480 mm Chipboard screws 4x15 L Top row R Top row LD drillings both.iam
- 560H_plus_Blumotion NL=480 mm Chipboard screws 4x15 L Top row R Top row LD drillings F.iam
- 560H_plus_Blumotion NL=480 mm Chipboard screws 4x15 L Top row R Top row LD drillings none.iam
- 560H_plus_Blumotion NL=480 mm Chipboard screws 661.1450.HG 6,3x14,5 L Bottom row R Bottom row LD drillings B.iam
- 560H_plus_Blumotion NL=480 mm Chipboard screws 661.1450.HG 6,3x14,5 L Bottom row R Bottom row LD drillings both.iam
- 560H_plus_Blumotion NL=480 mm Chipboard screws 661.1450.HG 6,3x14,5 L Bottom row R Bottom row LD drillings F.iam
- 560H_plus_Blumotion NL=480 mm Chipboard screws 661.1450.HG 6,3x14,5 L Bottom row R Bottom row LD drillings none.iam
- 560H_plus_Blumotion NL=480 mm Chipboard screws 661.1450.HG 6,3x14,5 L Bottom row R Top row LD drillings B.iam
- 560H_plus_Blumotion NL=480 mm Chipboard screws 661.1450.HG 6,3x14,5 L Bottom row R Top row LD drillings both.iam
- 560H_plus_Blumotion NL=480 mm Chipboard screws 661.1450.HG 6,3x14,5 L Bottom row R Top row LD drillings F.iam
- 560H_plus_Blumotion NL=480 mm Chipboard screws 661.1450.HG 6,3x14,5 L Bottom row R Top row LD drillings none.iam
- 560H_plus_Blumotion NL=480 mm Chipboard screws 661.1450.HG 6,3x14,5 L Top row R Bottom row LD drillings B.iam
- 560H_plus_Blumotion NL=480 mm Chipboard screws 661.1450.HG 6,3x14,5 L Top row R Bottom row LD drillings both.iam
- 560H_plus_Blumotion NL=480 mm Chipboard screws 661.1450.HG 6,3x14,5 L Top row R Bottom row LD drillings F.iam
- 560H_plus_Blumotion NL=480 mm Chipboard screws 661.1450.HG 6,3x14,5 L Top row R Bottom row LD drillings none.iam
- 560H_plus_Blumotion NL=480 mm Chipboard screws 661.1450.HG 6,3x14,5 L Top row R Top row LD drillings B.iam
- 560H_plus_Blumotion NL=480 mm Chipboard screws 661.1450.HG 6,3x14,5 L Top row R Top row LD drillings both.iam
- 560H_plus_Blumotion NL=480 mm Chipboard screws 661.1450.HG 6,3x14,5 L Top row R Top row LD drillings F.iam
- 560H_plus_Blumotion NL=480 mm Chipboard screws 661.1450.HG 6,3x14,5 L Top row R Top row LD drillings none.iam
- 560H_plus_Blumotion NL=500 mm Chipboard screws 4x15 L Bottom row R Bottom row LD drillings B.iam
- 560H_plus_Blumotion NL=500 mm Chipboard screws 4x15 L Bottom row R Bottom row LD drillings both.iam
- 560H_plus_Blumotion NL=500 mm Chipboard screws 4x15 L Bottom row R Bottom row LD drillings F.iam
- 560H_plus_Blumotion NL=500 mm Chipboard screws 4x15 L Bottom row R Bottom row LD drillings none.iam
- 560H_plus_Blumotion NL=500 mm Chipboard screws 4x15 L Bottom row R Top row LD drillings B.iam
- 560H_plus_Blumotion NL=500 mm Chipboard screws 4x15 L Bottom row R Top row LD drillings both.iam
- 560H_plus_Blumotion NL=500 mm Chipboard screws 4x15 L Bottom row R Top row LD drillings F.iam
- 560H_plus_Blumotion NL=500 mm Chipboard screws 4x15 L Bottom row R Top row LD drillings none.iam
- 560H_plus_Blumotion NL=500 mm Chipboard screws 4x15 L Top row R Bottom row LD drillings B.iam
- 560H_plus_Blumotion NL=500 mm Chipboard screws 4x15 L Top row R Bottom row LD drillings both.iam
- 560H_plus_Blumotion NL=500 mm Chipboard screws 4x15 L Top row R Bottom row LD drillings F.iam
- 560H_plus_Blumotion NL=500 mm Chipboard screws 4x15 L Top row R Bottom row LD drillings none.iam
- 560H_plus_Blumotion NL=500 mm Chipboard screws 4x15 L Top row R Top row LD drillings B.iam
- 560H_plus_Blumotion NL=500 mm Chipboard screws 4x15 L Top row R Top row LD drillings both.iam
- 560H_plus_Blumotion NL=500 mm Chipboard screws 4x15 L Top row R Top row LD drillings F.iam
- 560H_plus_Blumotion NL=500 mm Chipboard screws 4x15 L Top row R Top row LD drillings none.iam
- 560H_plus_Blumotion NL=500 mm Chipboard screws 661.1450.HG 6,3x14,5 L Bottom row R Bottom row LD drillings B.iam
- 560H_plus_Blumotion NL=500 mm Chipboard screws 661.1450.HG 6,3x14,5 L Bottom row R Bottom row LD drillings both.iam
- 560H_plus_Blumotion NL=500 mm Chipboard screws 661.1450.HG 6,3x14,5 L Bottom row R Bottom row LD drillings F.iam
- 560H_plus_Blumotion NL=500 mm Chipboard screws 661.1450.HG 6,3x14,5 L Bottom row R Bottom row LD drillings none.iam
- 560H_plus_Blumotion NL=500 mm Chipboard screws 661.1450.HG 6,3x14,5 L Bottom row R Top row LD drillings B.iam
- 560H_plus_Blumotion NL=500 mm Chipboard screws 661.1450.HG 6,3x14,5 L Bottom row R Top row LD drillings both.iam
- 560H_plus_Blumotion NL=500 mm Chipboard screws 661.1450.HG 6,3x14,5 L Bottom row R Top row LD drillings F.iam
- 560H_plus_Blumotion NL=500 mm Chipboard screws 661.1450.HG 6,3x14,5 L Bottom row R Top row LD drillings none.iam
- 560H_plus_Blumotion NL=500 mm Chipboard screws 661.1450.HG 6,3x14,5 L Top row R Bottom row LD drillings B.iam
- 560H_plus_Blumotion NL=500 mm Chipboard screws 661.1450.HG 6,3x14,5 L Top row R Bottom row LD drillings both.iam
- 560H_plus_Blumotion NL=500 mm Chipboard screws 661.1450.HG 6,3x14,5 L Top row R Bottom row LD drillings F.iam
- 560H_plus_Blumotion NL=500 mm Chipboard screws 661.1450.HG 6,3x14,5 L Top row R Bottom row LD drillings none.iam
- 560H_plus_Blumotion NL=500 mm Chipboard screws 661.1450.HG 6,3x14,5 L Top row R Top row LD drillings B.iam
- 560H_plus_Blumotion NL=500 mm Chipboard screws 661.1450.HG 6,3x14,5 L Top row R Top row LD drillings both.iam
- 560H_plus_Blumotion NL=500 mm Chipboard screws 661.1450.HG 6,3x14,5 L Top row R Top row LD drillings F.iam
- 560H_plus_Blumotion NL=500 mm Chipboard screws 661.1450.HG 6,3x14,5 L Top row R Top row LD drillings none.iam
- 560H_plus_Blumotion NL=520 mm Chipboard screws 4x15 L Bottom row R Bottom row LD drillings B.iam
- 560H_plus_Blumotion NL=520 mm Chipboard screws 4x15 L Bottom row R Bottom row LD drillings both.iam
- 560H_plus_Blumotion NL=520 mm Chipboard screws 4x15 L Bottom row R Bottom row LD drillings F.iam
- 560H_plus_Blumotion NL=520 mm Chipboard screws 4x15 L Bottom row R Bottom row LD drillings none.iam
- 560H_plus_Blumotion NL=520 mm Chipboard screws 4x15 L Bottom row R Top row LD drillings B.iam
- 560H_plus_Blumotion NL=520 mm Chipboard screws 4x15 L Bottom row R Top row LD drillings both.iam
- 560H_plus_Blumotion NL=520 mm Chipboard screws 4x15 L Bottom row R Top row LD drillings F.iam
- 560H_plus_Blumotion NL=520 mm Chipboard screws 4x15 L Bottom row R Top row LD drillings none.iam
- 560H_plus_Blumotion NL=520 mm Chipboard screws 4x15 L Top row R Bottom row LD drillings B.iam
- 560H_plus_Blumotion NL=520 mm Chipboard screws 4x15 L Top row R Bottom row LD drillings both.iam
- 560H_plus_Blumotion NL=520 mm Chipboard screws 4x15 L Top row R Bottom row LD drillings F.iam
- 560H_plus_Blumotion NL=520 mm Chipboard screws 4x15 L Top row R Bottom row LD drillings none.iam
- 560H_plus_Blumotion NL=520 mm Chipboard screws 4x15 L Top row R Top row LD drillings B.iam
- 560H_plus_Blumotion NL=520 mm Chipboard screws 4x15 L Top row R Top row LD drillings both.iam
- 560H_plus_Blumotion NL=520 mm Chipboard screws 4x15 L Top row R Top row LD drillings F.iam
- 560H_plus_Blumotion NL=520 mm Chipboard screws 4x15 L Top row R Top row LD drillings none.iam
- 560H_plus_Blumotion NL=520 mm Chipboard screws 661.1450.HG 6,3x14,5 L Bottom row R Bottom row LD drillings B.iam
- 560H_plus_Blumotion NL=520 mm Chipboard screws 661.1450.HG 6,3x14,5 L Bottom row R Bottom row LD drillings both.iam
- 560H_plus_Blumotion NL=520 mm Chipboard screws 661.1450.HG 6,3x14,5 L Bottom row R Bottom row LD drillings F.iam
- 560H_plus_Blumotion NL=520 mm Chipboard screws 661.1450.HG 6,3x14,5 L Bottom row R Bottom row LD drillings none.iam
- 560H_plus_Blumotion NL=520 mm Chipboard screws 661.1450.HG 6,3x14,5 L Bottom row R Top row LD drillings B.iam
- 560H_plus_Blumotion NL=520 mm Chipboard screws 661.1450.HG 6,3x14,5 L Bottom row R Top row LD drillings both.iam
- 560H_plus_Blumotion NL=520 mm Chipboard screws 661.1450.HG 6,3x14,5 L Bottom row R Top row LD drillings F.iam
- 560H_plus_Blumotion NL=520 mm Chipboard screws 661.1450.HG 6,3x14,5 L Bottom row R Top row LD drillings none.iam
- 560H_plus_Blumotion NL=520 mm Chipboard screws 661.1450.HG 6,3x14,5 L Top row R Bottom row LD drillings B.iam
- 560H_plus_Blumotion NL=520 mm Chipboard screws 661.1450.HG 6,3x14,5 L Top row R Bottom row LD drillings both.iam
- 560H_plus_Blumotion NL=520 mm Chipboard screws 661.1450.HG 6,3x14,5 L Top row R Bottom row LD drillings F.iam
- 560H_plus_Blumotion NL=520 mm Chipboard screws 661.1450.HG 6,3x14,5 L Top row R Bottom row LD drillings none.iam
- 560H_plus_Blumotion NL=520 mm Chipboard screws 661.1450.HG 6,3x14,5 L Top row R Top row LD drillings B.iam
- 560H_plus_Blumotion NL=520 mm Chipboard screws 661.1450.HG 6,3x14,5 L Top row R Top row LD drillings both.iam
- 560H_plus_Blumotion NL=520 mm Chipboard screws 661.1450.HG 6,3x14,5 L Top row R Top row LD drillings F.iam
- 560H_plus_Blumotion NL=520 mm Chipboard screws 661.1450.HG 6,3x14,5 L Top row R Top row LD drillings none.iam
- 560H_plus_Blumotion NL=550 mm Chipboard screws 4x15 L Bottom row R Bottom row LD drillings B.iam
- 560H_plus_Blumotion NL=550 mm Chipboard screws 4x15 L Bottom row R Bottom row LD drillings both.iam
- 560H_plus_Blumotion NL=550 mm Chipboard screws 4x15 L Bottom row R Bottom row LD drillings F.iam
- 560H_plus_Blumotion NL=550 mm Chipboard screws 4x15 L Bottom row R Bottom row LD drillings none.iam
- 560H_plus_Blumotion NL=550 mm Chipboard screws 4x15 L Bottom row R Top row LD drillings B.iam
- 560H_plus_Blumotion NL=550 mm Chipboard screws 4x15 L Bottom row R Top row LD drillings both.iam
- 560H_plus_Blumotion NL=550 mm Chipboard screws 4x15 L Bottom row R Top row LD drillings F.iam
- 560H_plus_Blumotion NL=550 mm Chipboard screws 4x15 L Bottom row R Top row LD drillings none.iam
- 560H_plus_Blumotion NL=550 mm Chipboard screws 4x15 L Top row R Bottom row LD drillings B.iam
- 560H_plus_Blumotion NL=550 mm Chipboard screws 4x15 L Top row R Bottom row LD drillings both.iam
- 560H_plus_Blumotion NL=550 mm Chipboard screws 4x15 L Top row R Bottom row LD drillings F.iam
- 560H_plus_Blumotion NL=550 mm Chipboard screws 4x15 L Top row R Bottom row LD drillings none.iam
- 560H_plus_Blumotion NL=550 mm Chipboard screws 4x15 L Top row R Top row LD drillings B.iam
- 560H_plus_Blumotion NL=550 mm Chipboard screws 4x15 L Top row R Top row LD drillings both.iam
- 560H_plus_Blumotion NL=550 mm Chipboard screws 4x15 L Top row R Top row LD drillings F.iam
- 560H_plus_Blumotion NL=550 mm Chipboard screws 4x15 L Top row R Top row LD drillings none.iam
- 560H_plus_Blumotion NL=550 mm Chipboard screws 661.1450.HG 6,3x14,5 L Bottom row R Bottom row LD drillings B.iam
- 560H_plus_Blumotion NL=550 mm Chipboard screws 661.1450.HG 6,3x14,5 L Bottom row R Bottom row LD drillings both.iam
- 560H_plus_Blumotion NL=550 mm Chipboard screws 661.1450.HG 6,3x14,5 L Bottom row R Bottom row LD drillings F.iam
- 560H_plus_Blumotion NL=550 mm Chipboard screws 661.1450.HG 6,3x14,5 L Bottom row R Bottom row LD drillings none.iam
- 560H_plus_Blumotion NL=550 mm Chipboard screws 661.1450.HG 6,3x14,5 L Bottom row R Top row LD drillings B.iam
- 560H_plus_Blumotion NL=550 mm Chipboard screws 661.1450.HG 6,3x14,5 L Bottom row R Top row LD drillings both.iam
- 560H_plus_Blumotion NL=550 mm Chipboard screws 661.1450.HG 6,3x14,5 L Bottom row R Top row LD drillings F.iam
- 560H_plus_Blumotion NL=550 mm Chipboard screws 661.1450.HG 6,3x14,5 L Bottom row R Top row LD drillings none.iam
- 560H_plus_Blumotion NL=550 mm Chipboard screws 661.1450.HG 6,3x14,5 L Top row R Bottom row LD drillings B.iam
- 560H_plus_Blumotion NL=550 mm Chipboard screws 661.1450.HG 6,3x14,5 L Top row R Bottom row LD drillings both.iam
- 560H_plus_Blumotion NL=550 mm Chipboard screws 661.1450.HG 6,3x14,5 L Top row R Bottom row LD drillings F.iam
- 560H_plus_Blumotion NL=550 mm Chipboard screws 661.1450.HG 6,3x14,5 L Top row R Bottom row LD drillings none.iam
- 560H_plus_Blumotion NL=550 mm Chipboard screws 661.1450.HG 6,3x14,5 L Top row R Top row LD drillings B.iam
- 560H_plus_Blumotion NL=550 mm Chipboard screws 661.1450.HG 6,3x14,5 L Top row R Top row LD drillings both.iam
- 560H_plus_Blumotion NL=550 mm Chipboard screws 661.1450.HG 6,3x14,5 L Top row R Top row LD drillings F.iam
- 560H_plus_Blumotion NL=550 mm Chipboard screws 661.1450.HG 6,3x14,5 L Top row R Top row LD drillings none.iam
- 560H_plus_Blumotion NL=600 mm Chipboard screws 4x15 L Bottom row R Bottom row LD drillings B.iam
- 560H_plus_Blumotion NL=600 mm Chipboard screws 4x15 L Bottom row R Bottom row LD drillings both.iam
- 560H_plus_Blumotion NL=600 mm Chipboard screws 4x15 L Bottom row R Bottom row LD drillings F.iam
- 560H_plus_Blumotion NL=600 mm Chipboard screws 4x15 L Bottom row R Bottom row LD drillings none.iam
- 560H_plus_Blumotion NL=600 mm Chipboard screws 4x15 L Bottom row R Top row LD drillings B.iam
- 560H_plus_Blumotion NL=600 mm Chipboard screws 4x15 L Bottom row R Top row LD drillings both.iam
- 560H_plus_Blumotion NL=600 mm Chipboard screws 4x15 L Bottom row R Top row LD drillings F.iam
- 560H_plus_Blumotion NL=600 mm Chipboard screws 4x15 L Bottom row R Top row LD drillings none.iam
- 560H_plus_Blumotion NL=600 mm Chipboard screws 4x15 L Top row R Bottom row LD drillings B.iam
- 560H_plus_Blumotion NL=600 mm Chipboard screws 4x15 L Top row R Bottom row LD drillings both.iam
- 560H_plus_Blumotion NL=600 mm Chipboard screws 4x15 L Top row R Bottom row LD drillings F.iam
- 560H_plus_Blumotion NL=600 mm Chipboard screws 4x15 L Top row R Bottom row LD drillings none.iam
- 560H_plus_Blumotion NL=600 mm Chipboard screws 4x15 L Top row R Top row LD drillings B.iam
- 560H_plus_Blumotion NL=600 mm Chipboard screws 4x15 L Top row R Top row LD drillings both.iam
- 560H_plus_Blumotion NL=600 mm Chipboard screws 4x15 L Top row R Top row LD drillings F.iam
- 560H_plus_Blumotion NL=600 mm Chipboard screws 4x15 L Top row R Top row LD drillings none.iam
- 560H_plus_Blumotion NL=600 mm Chipboard screws 661.1450.HG 6,3x14,5 L Bottom row R Bottom row LD drillings B.iam
- 560H_plus_Blumotion NL=600 mm Chipboard screws 661.1450.HG 6,3x14,5 L Bottom row R Bottom row LD drillings both.iam
- 560H_plus_Blumotion NL=600 mm Chipboard screws 661.1450.HG 6,3x14,5 L Bottom row R Bottom row LD drillings F.iam
- 560H_plus_Blumotion NL=600 mm Chipboard screws 661.1450.HG 6,3x14,5 L Bottom row R Bottom row LD drillings none.iam
- 560H_plus_Blumotion NL=600 mm Chipboard screws 661.1450.HG 6,3x14,5 L Bottom row R Top row LD drillings B.iam
- 560H_plus_Blumotion NL=600 mm Chipboard screws 661.1450.HG 6,3x14,5 L Bottom row R Top row LD drillings both.iam
- 560H_plus_Blumotion NL=600 mm Chipboard screws 661.1450.HG 6,3x14,5 L Bottom row R Top row LD drillings F.iam
- 560H_plus_Blumotion NL=600 mm Chipboard screws 661.1450.HG 6,3x14,5 L Bottom row R Top row LD drillings none.iam
- 560H_plus_Blumotion NL=600 mm Chipboard screws 661.1450.HG 6,3x14,5 L Top row R Bottom row LD drillings B.iam
- 560H_plus_Blumotion NL=600 mm Chipboard screws 661.1450.HG 6,3x14,5 L Top row R Bottom row LD drillings both.iam
- 560H_plus_Blumotion NL=600 mm Chipboard screws 661.1450.HG 6,3x14,5 L Top row R Bottom row LD drillings F.iam
- 560H_plus_Blumotion NL=600 mm Chipboard screws 661.1450.HG 6,3x14,5 L Top row R Bottom row LD drillings none.iam
- 560H_plus_Blumotion NL=600 mm Chipboard screws 661.1450.HG 6,3x14,5 L Top row R Top row LD drillings B.iam
- 560H_plus_Blumotion NL=600 mm Chipboard screws 661.1450.HG 6,3x14,5 L Top row R Top row LD drillings both.iam
- 560H_plus_Blumotion NL=600 mm Chipboard screws 661.1450.HG 6,3x14,5 L Top row R Top row LD drillings F.iam
- 560H_plus_Blumotion NL=600 mm Chipboard screws 661.1450.HG 6,3x14,5 L Top row R Top row LD drillings none.iam
- C:\Users\Public\Documents\Woodwork for Inventor\Textures\Black.png
## Components (4 placed, 4 different names)
1. 560H2700B Chipboard screws top_row L:1 — Flush:1, Flush:2, Flush:7, Flush:5
2. 560H2700B Chipboard screws top_row R:2 — Flush:1, Flush:2, Flush:8, Flush:6
3. Locking device L:1 — Flush:7, Flush:3, Flush:4, Flush:5
4. Locking device R:2 — Flush:8, Flush:3, Flush:4, Flush:6
## Relationships (8: Flush 8)
- Flush:1: 560H2700B Chipboard screws top_row L:1 ↔ 560H2700B Chipboard screws top_row R:2
- Flush:2: 560H2700B Chipboard screws top_row L:1 ↔ 560H2700B Chipboard screws top_row R:2
- Flush:7: 560H2700B Chipboard screws top_row L:1 ↔ Locking device L:1
- Flush:8: 560H2700B Chipboard screws top_row R:2 ↔ Locking device R:2
- Flush:3: Locking device L:1 ↔ Locking device R:2
- Flush:4: Locking device L:1 ↔ Locking device R:2
- Flush:5: 560H2700B Chipboard screws top_row L:1 ↔ Locking device L:1
- Flush:6 (-2 mm): 560H2700B Chipboard screws top_row R:2 ↔ Locking device R:2
